# Autodesk Inventor assembly: RailAttachmentAssemblyWithoutPi
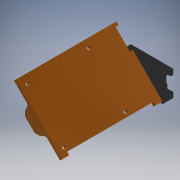
[picture p0: Inventor's stored thumbnail of the model, 180x180]
Saved by Autodesk Inventor 2018 (Build 220112000, 112)
## iProperties
Created: 2019-04-01
Part Number: RailAttachmentAssemblyWithoutPi
Document SubType Name: Assembly
Designer: snipe
Author: snipe
## Documents named in this file (3)
- C:\Users\snipe\Documents\CPRE186-CAD\RailAttachmentAssemblyWithoutPi.iam
- C:\Users\snipe\Documents\CPRE186-CAD\nerfRailMount.ipt
- C:\Users\snipe\Documents\CPRE186-CAD\Raspi3B+_Case.ipt
## Components (2 placed, 2 different names)
1. nerfRailMount:1 — Mate:1, Angle:1, Mate:4, Flush:1, Mate:6, Mate:7, Flush:2
2. Raspi3B+_Case:1 — Mate:1, Angle:1, Mate:6, Mate:7
## Relationships (7: Mate 4, Flush 2, Angle 1)
- Mate:1: nerfRailMount:1 ↔ Raspi3B+_Case:1
- Angle:1 (315 deg): nerfRailMount:1 ↔ Raspi3B+_Case:1
- Mate:4: nerfRailMount:1
- Flush:1: nerfRailMount:1
- Mate:6: nerfRailMount:1 ↔ Raspi3B+_Case:1
- Mate:7: nerfRailMount:1 ↔ Raspi3B+_Case:1
- Flush:2: nerfRailMount:1
